# Autodesk Inventor assembly: froggy prig assm
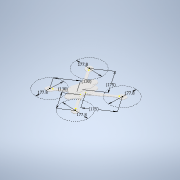
[picture p0: Inventor's stored thumbnail of the model, 180x180]
Saved by Autodesk Inventor 2020 (Build 240168000, 168)
## iProperties
Created: 2022-05-23
Part Number: froggy prig assm
Document SubType Name: Assembly
Designer: Steven
Author: Steven
## Documents named in this file (5)
- Y:\FPV drone stuff\0 Street League\Frames\experimental-quad-frames\froggy prig assm.iam
- Y:\FPV drone stuff\0 Street League\Frames\experimental-quad-frames\Kauri arm short.ipt
- Y:\FPV drone stuff\0 Street League\Frames\experimental-quad-frames\399 prig z plate.ipt
- Y:\FPV drone stuff\0 Street League\Frames\experimental-quad-frames\399 prig top plate.ipt
- Y:\FPV drone stuff\0 Street League\Frames\experimental-quad-frames\Kauri arm long.ipt
## Components (7 placed, 4 different names)
1. 399 prig z plate:1 — Mate:1, Mate:2, Mate:3, Mate:8, Mate:9, Mate:11, Mate:12, Insert:1, Mate:18
2. Kauri arm short:1 — Mate:1, Mate:2, Flush:3, Mate:3, Flush:4
3. Kauri arm short:4 — Flush:3, Mate:8, Mate:9, Mate:10, Flush:5
4. 399 prig z plate:2 — Mate:10, Mate:11, Mate:12, Mate:13, Mate:14, Mate:15, Mate:16, Mate:17
5. 399 prig top plate:1 — Mate:13, Mate:14, Mate:15
6. Kauri arm long:1 — Flush:4, Mate:17, Mate:18
7. Kauri arm long:2 — Flush:5, Insert:1, Mate:16
## Relationships (18: Mate 14, Flush 3, Insert 1)
- Mate:1: 399 prig z plate:1 ↔ Kauri arm short:1
- Mate:2: 399 prig z plate:1 ↔ Kauri arm short:1
- Flush:3: Kauri arm short:1 ↔ Kauri arm short:4
- Mate:3: 399 prig z plate:1 ↔ Kauri arm short:1
- Mate:8: 399 prig z plate:1 ↔ Kauri arm short:4
- Mate:9: 399 prig z plate:1 ↔ Kauri arm short:4
- Mate:10: Kauri arm short:4 ↔ 399 prig z plate:2
- Mate:11: 399 prig z plate:1 ↔ 399 prig z plate:2
- Mate:12: 399 prig z plate:1 ↔ 399 prig z plate:2
- Mate:13 (25 mm): 399 prig z plate:2 ↔ 399 prig top plate:1
- Mate:14: 399 prig z plate:2 ↔ 399 prig top plate:1
- Mate:15: 399 prig z plate:2 ↔ 399 prig top plate:1
- Flush:4: Kauri arm short:1 ↔ Kauri arm long:1
- Flush:5: Kauri arm short:4 ↔ Kauri arm long:2
- Insert:1: 399 prig z plate:1 ↔ Kauri arm long:2
- Mate:16: 399 prig z plate:2 ↔ Kauri arm long:2
- Mate:17: 399 prig z plate:2 ↔ Kauri arm long:1
- Mate:18: 399 prig z plate:1 ↔ Kauri arm long:1
